# Autodesk Inventor assembly: NewMechanumWheelSubAssembly
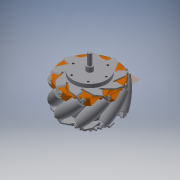
[picture p0: Inventor's stored thumbnail of the model, 180x180]
Saved by Autodesk Inventor 2017 (Build 210142000, 142)
## iProperties
Created: 2017-08-16
Part Number: NewMechanumWheelSubAssembly
Document SubType Name: Assembly
Designer: User
Author: User
## Documents named in this file (6)
- C:\Robotics\CAD\2016-17_CAD\DriveTrain\NewMechanumWheelSubAssembly.iam
- C:\Robotics\CAD\2016-17_CAD\Mecanum Wheel Adapter Plate.ipt
- C:\Robotics\CAD\COTSParts\Actobotics\615 parts\615106.ipt
- C:\Robotics\CAD\COTSParts\Actobotics\634 parts\634080.ipt
- C:\Robotics\CAD\COTSParts\Wheels\AndyMark Mecanum Wheels\100mm Aluminum Mecanum wheels.ipt
- C:\Robotics\CAD\2016-17_CAD\Mecanum Wheel Adapter.ipt
## Components (5 placed, 5 different names)
1. Mecanum Wheel Adapter Plate:1 — Mate:1, Mate:2, Mate:5, Flush:1
2. 615106:1 — Mate:3, Mate:4
3. 634080:1 — Mate:5, Flush:1
4. 100mm Aluminum Mecanum wheels:1 — Insert:1, Mate:1, Mate:2
5. Mecanum Wheel Adapter:1 — Insert:1, Mate:3, Mate:4
## Relationships (7: Mate 5, Insert 1, Flush 1)
- Insert:1: 100mm Aluminum Mecanum wheels:1 ↔ Mecanum Wheel Adapter:1
- Mate:1: Mecanum Wheel Adapter Plate:1 ↔ 100mm Aluminum Mecanum wheels:1
- Mate:2: Mecanum Wheel Adapter Plate:1 ↔ 100mm Aluminum Mecanum wheels:1
- Mate:3 (6.35 mm): 615106:1 ↔ Mecanum Wheel Adapter:1
- Mate:4: 615106:1 ↔ Mecanum Wheel Adapter:1
- Mate:5: Mecanum Wheel Adapter Plate:1 ↔ 634080:1
- Flush:1 (-18.2118 mm): Mecanum Wheel Adapter Plate:1 ↔ 634080:1
